# Autodesk Inventor assembly: back
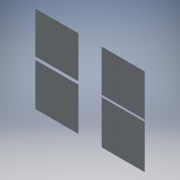
[picture p0: Inventor's stored thumbnail of the model, 180x180]
Saved by Autodesk Inventor 2019 (Build 230136000, 136)
## iProperties
Created: 2018-07-10
Part Number: back
Document SubType Name: Assembly
Designer: User
Author: User
## Documents named in this file (5)
- C:\Users\User\Desktop\Room Model\back.iam
- C:\Users\User\Desktop\Room Model\back_0_0.ipt
- C:\Users\User\Desktop\Room Model\back_0_1.ipt
- C:\Users\User\Desktop\Room Model\back_1_0.ipt
- C:\Users\User\Desktop\Room Model\back_1_1.ipt
## Components (4 placed, 4 different names)
1. back_0_0:1 — Rigid:1, Rigid:2
2. back_0_1:1 — Rigid:1
3. back_1_0:1 — Rigid:2, Rigid:3
4. back_1_1:1 — Rigid:3
## Relationships (3: WeldJoint 3)
- Rigid:1 [WeldJoint] (660.4 mm): back_0_0:1 ↔ back_0_1:1
- Rigid:2 [WeldJoint] (82.55 mm): back_0_0:1 ↔ back_1_0:1
- Rigid:3 [WeldJoint] (660.4 mm): back_1_0:1 ↔ back_1_1:1
